# Autodesk Inventor assembly: frame assembly 7
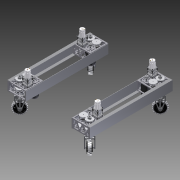
[picture p0: Inventor's stored thumbnail of the model, 180x180]
Saved by Autodesk Inventor 2012 (Build 160160000, 160)
## iProperties
Created: 2013-07-20
Part Number: frame assembly 7
Document SubType Name: Assembly
Designer: Bryce
Author: Bryce
## Documents named in this file (4)
- C:\Users\Bryce\Dropbox\Inventor Design Project Files\Independent Swerves\Inventor 2012\frame assembly 7.iam
- C:\Users\Bryce\Dropbox\Inventor Design Project Files\Independent Swerves\Inventor 2012\FULL SWERVE DRIVE ASSEMBLY!  2!.iam
- C:\Users\Bryce\Dropbox\Inventor Design Project Files\Independent Swerves\Inventor 2012\frame 7 outside U.ipt
- C:\Users\Bryce\Dropbox\Inventor Design Project Files\Independent Swerves\Inventor 2012\frame 7 inside L.ipt
## Components (8 placed, 3 different names)
1. FULL SWERVE DRIVE ASSEMBLY!  2!:1 [sub-assembly] — Mate:1, Flush:1, Mate:2, Flush:3, Flush:6, Flush:8, Mate:7, Flush:11, Mate:9
2. FULL SWERVE DRIVE ASSEMBLY!  2!:2 [sub-assembly] — Flush:3, Flush:4, Flush:7, Flush:8
3. FULL SWERVE DRIVE ASSEMBLY!  2!:3 [sub-assembly] — Flush:4, Flush:5, Flush:7, Flush:9, Flush:10, Mate:6
4. FULL SWERVE DRIVE ASSEMBLY!  2!:4 [sub-assembly] — Mate:3, Mate:4, Flush:2, Flush:5, Flush:6, Flush:9, Flush:12, Mate:8
5. frame 7 outside U:1 — Mate:1, Flush:1, Mate:2, Mate:5
6. frame 7 outside U:2 — Mate:3, Mate:4, Flush:2, Mate:5, Flush:10
7. frame 7 inside L:1 — Mate:7, Flush:11, Mate:9
8. frame 7 inside L:2 — Mate:6, Flush:12, Mate:8
## Relationships (21: Flush 12, Mate 9)
- Mate:1: FULL SWERVE DRIVE ASSEMBLY!  2!:1 ↔ frame 7 outside U:1
- Flush:1: FULL SWERVE DRIVE ASSEMBLY!  2!:1 ↔ frame 7 outside U:1
- Mate:2: FULL SWERVE DRIVE ASSEMBLY!  2!:1 ↔ frame 7 outside U:1
- Mate:3: FULL SWERVE DRIVE ASSEMBLY!  2!:4 ↔ frame 7 outside U:2
- Mate:4: FULL SWERVE DRIVE ASSEMBLY!  2!:4 ↔ frame 7 outside U:2
- Flush:2: FULL SWERVE DRIVE ASSEMBLY!  2!:4 ↔ frame 7 outside U:2
- Flush:3: FULL SWERVE DRIVE ASSEMBLY!  2!:1 ↔ FULL SWERVE DRIVE ASSEMBLY!  2!:2
- Flush:4: FULL SWERVE DRIVE ASSEMBLY!  2!:2 ↔ FULL SWERVE DRIVE ASSEMBLY!  2!:3
- Flush:5: FULL SWERVE DRIVE ASSEMBLY!  2!:3 ↔ FULL SWERVE DRIVE ASSEMBLY!  2!:4
- Flush:6: FULL SWERVE DRIVE ASSEMBLY!  2!:1 ↔ FULL SWERVE DRIVE ASSEMBLY!  2!:4
- Flush:7: FULL SWERVE DRIVE ASSEMBLY!  2!:2 ↔ FULL SWERVE DRIVE ASSEMBLY!  2!:3
- Flush:8: FULL SWERVE DRIVE ASSEMBLY!  2!:1 ↔ FULL SWERVE DRIVE ASSEMBLY!  2!:2
- Flush:9: FULL SWERVE DRIVE ASSEMBLY!  2!:3 ↔ FULL SWERVE DRIVE ASSEMBLY!  2!:4
- Mate:5 (-711.2 mm): frame 7 outside U:1 ↔ frame 7 outside U:2
- Flush:10: FULL SWERVE DRIVE ASSEMBLY!  2!:3 ↔ frame 7 outside U:2
- Mate:6: FULL SWERVE DRIVE ASSEMBLY!  2!:3 ↔ frame 7 inside L:2
- Mate:7: FULL SWERVE DRIVE ASSEMBLY!  2!:1 ↔ frame 7 inside L:1
- Flush:11: FULL SWERVE DRIVE ASSEMBLY!  2!:1 ↔ frame 7 inside L:1
- Flush:12: FULL SWERVE DRIVE ASSEMBLY!  2!:4 ↔ frame 7 inside L:2
- Mate:8: FULL SWERVE DRIVE ASSEMBLY!  2!:4 ↔ frame 7 inside L:2
- Mate:9: FULL SWERVE DRIVE ASSEMBLY!  2!:1 ↔ frame 7 inside L:1
